# Autodesk Inventor assembly: Kettenantrieb
Saved by Autodesk Inventor 2016 (Build 200138000, 138)
## iProperties
Created: 2017-12-11
Part Number: Kettenantrieb
Document SubType Name: Assembly
Designer: Dominik
ClientObjectVersion: 1
Author: Dominik
## Documents named in this file (4)
- C:\Users\Dominik\Desktop\Diplomarbeit\fuettr_prototype\Mechanical\Inventorskizzen\Plattenzusammensetzung\Konstruktions-Assistent\Kettenantrieb1.iam
- C:\Users\Dominik\Desktop\Diplomarbeit\fuettr_prototype\Mechanical\Inventorskizzen\Plattenzusammensetzung\Konstruktions-Assistent\Rollenkette1.ipt
- C:\Users\Dominik\Desktop\Diplomarbeit\fuettr_prototype\Mechanical\Inventorskizzen\Plattenzusammensetzung\Konstruktions-Assistent\Kettenrad der Rollenkette11.ipt
- C:\Users\Dominik\Desktop\Diplomarbeit\fuettr_prototype\Mechanical\Inventorskizzen\Plattenzusammensetzung\Konstruktions-Assistent\Kettenrad der Rollenkette21.ipt
## Components (3 placed, 3 different names)
1. Rollenkette:1 — Fluchtend:1, Fluchtend:2
2. Kettenrad der Rollenkette1:1 — Fluchtend:1, Drehung:1
3. Kettenrad der Rollenkette2:1 — Fluchtend:2, Drehung:1
## Relationships (3: Flush 2, RelateRotation 1)
- Fluchtend:1 [Flush]: Rollenkette:1 ↔ Kettenrad der Rollenkette1:1
- Fluchtend:2 [Flush]: Rollenkette:1 ↔ Kettenrad der Rollenkette2:1
- Drehung:1 [RelateRotation] (3 ul): Kettenrad der Rollenkette1:1 ↔ Kettenrad der Rollenkette2:1
